# Autodesk Inventor assembly: Assembly6
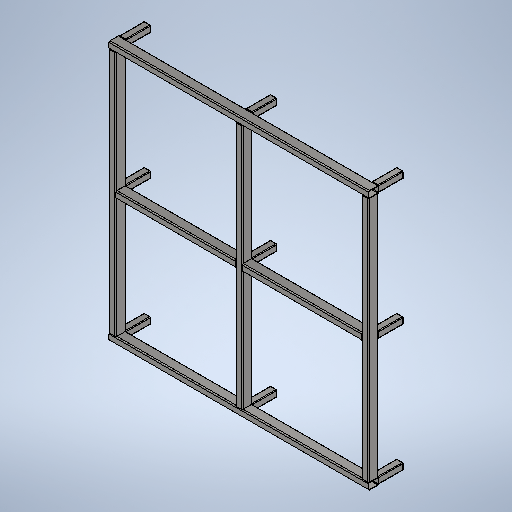
[picture p0: Inventor's stored thumbnail of the model, 512x512]
Saved by Autodesk Inventor 2025 (Build 290162010, 162A)
## iProperties
Created: 2024-09-20
Part Number: Assembly6
Document SubType Name: Assembly
Designer: admin
Author: admin
## Documents named in this file (3)
- C:\Users\admin\YandexDisk-badmisterfox\домашниий пк\Inventor\BSH_Beshkino_bio_tank\Assembly6.iam
- C:\Users\admin\YandexDisk-badmisterfox\домашниий пк\Inventor\BSH_Beshkino_bio_tank\Тумба 4.iam
- C:\Users\admin\YandexDisk-badmisterfox\домашниий пк\Inventor\BSH_Beshkino_bio_tank\ISO 4019 - 40x40x2 - 140.ipt
## Components (10 placed, 2 different names)
1. Тумба 4:1 [sub-assembly] — Rigid:1
2. ISO 4019 - 40x40x2 - 140:1 — Rigid:1
3. ISO 4019 - 40x40x2 - 140:2
4. ISO 4019 - 40x40x2 - 140:3
5. ISO 4019 - 40x40x2 - 140:4
6. ISO 4019 - 40x40x2 - 140:5
7. ISO 4019 - 40x40x2 - 140:6
8. ISO 4019 - 40x40x2 - 140:7
9. ISO 4019 - 40x40x2 - 140:8
10. ISO 4019 - 40x40x2 - 140:9
## Component patterns: (9 elements, first: ISO 4019 - 40x40x2 - 140:1)
## Relationships (1: WeldJoint 1)
- Rigid:1 [WeldJoint]: Тумба 4:1 ↔ ISO 4019 - 40x40x2 - 140:1
